# Autodesk Inventor assembly: SCARA
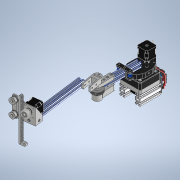
[picture p0: Inventor's stored thumbnail of the model, 180x180]
Saved by Autodesk Inventor 2022 (Build 260153000, 153)
## iProperties
Created: 2022-03-02
Part Number: SCARA
Document SubType Name: Assembly
Designer: JK
Author: JK
## Documents named in this file (5)
- C:\Users\JK\Documents\Inventor\ScaraNema\SCARA-3DP\Parts\SCARA.iam
- C:\Users\JK\Documents\Inventor\ScaraNema\SCARA-3DP\Parts\Shoulder\Shoulder base.iam
- C:\Users\JK\Documents\Inventor\ScaraNema\SCARA-3DP\Parts\Elbow\Elbow assembly.iam
- C:\Users\JK\Documents\Inventor\ScaraNema\SCARA-3DP\Parts\Z axis\Z assembly.iam
- C:\Users\JK\Documents\Inventor\ScaraNema\SCARA-3DP\Parts\Electronics\Electronics.iam
## Components (4 placed, 4 different names)
1. Shoulder base:1 [sub-assembly] — Coincidencia:3, Ángulo:1, Coincidencia:4
2. Elbow assembly:1 [sub-assembly]
3. Z assembly:1 [sub-assembly]
4. Electronics:1 [sub-assembly] — Coincidencia:3, Ángulo:1, Coincidencia:4
## Relationships (3: Mate 2, Angle 1)
- Coincidencia:3 [Mate]: Shoulder base:1 ↔ Electronics:1
- Ángulo:1 [Angle] (0 deg): Shoulder base:1 ↔ Electronics:1
- Coincidencia:4 [Mate]: Shoulder base:1 ↔ Electronics:1
